# Autodesk Inventor assembly: RescueKitThrow_Slope
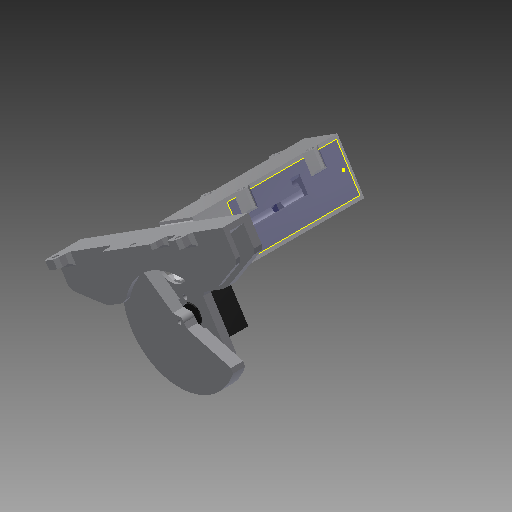
[picture p0: Inventor's stored thumbnail of the model, 512x512]
Saved by Autodesk Inventor 2018.3 (Build 223284000, 284)
## iProperties
Created: 2019-02-16
Part Number: RescueKitThrow_Slope
Material: 一般
Document SubType Name: Assembly
Designer: shun2
Author: shun2
## Documents named in this file (5)
- C:\Users\shun2\OneDrive\おそらく最新版(2018.7.31)\レスキューキット投下機構\RescueKitThrow_Slope.iam
- C:\Users\shun2\OneDrive\おそらく最新版(2018.7.31)\レスキューキット投下機構\RescueKitThrow_pipe.ipt
- C:\Users\shun2\OneDrive\おそらく最新版(2018.7.31)\レスキューキット投下機構\RescueKitThrow_slope.ipt
- C:\Users\shun2\OneDrive\おそらく最新版(2018.7.31)\レスキューキット投下機構\RescueKitThrow-Joint.ipt
- C:\Users\shun2\OneDrive\おそらく最新版(2018.7.31)\レスキューキット投下機構\RB-001-Servo.ipt
## Components (4 placed, 4 different names)
1. RescueKitThrow_pipe:1 — メイト:9, メイト:12, メイト:13, メイト:14
2. RescueKitThrow-Joint:1 — メイト:6, メイト:7
3. RescueKitThrow_slope:1 — メイト:8, メイト:9, メイト:10, メイト:11, メイト:12, メイト:13, メイト:14
4. RB-001-Servo:1 — メイト:6, メイト:7, メイト:8, メイト:10, メイト:11
## Relationships (9: Mate 9)
- メイト:6 [Mate]: RescueKitThrow-Joint:1 ↔ RB-001-Servo:1
- メイト:7 [Mate] (1 mm): RescueKitThrow-Joint:1 ↔ RB-001-Servo:1
- メイト:8 [Mate] (-3 mm): RescueKitThrow_slope:1 ↔ RB-001-Servo:1
- メイト:9 [Mate]: RescueKitThrow_pipe:1 ↔ RescueKitThrow_slope:1
- メイト:10 [Mate]: RescueKitThrow_slope:1 ↔ RB-001-Servo:1
- メイト:11 [Mate]: RescueKitThrow_slope:1 ↔ RB-001-Servo:1
- メイト:12 [Mate]: RescueKitThrow_pipe:1 ↔ RescueKitThrow_slope:1
- メイト:13 [Mate] (0.5 mm): RescueKitThrow_pipe:1 ↔ RescueKitThrow_slope:1
- メイト:14 [Mate] (0.5 mm): RescueKitThrow_pipe:1 ↔ RescueKitThrow_slope:1
